# Autodesk Inventor assembly: Robot
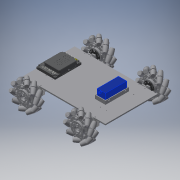
[picture p0: Inventor's stored thumbnail of the model, 180x180]
Saved by Autodesk Inventor 2017 (Build 210142000, 142)
## iProperties
Created: 2017-09-30
Part Number: Robot
Document SubType Name: Assembly
Designer: User
Author: User
## Documents named in this file (6)
- C:\Robotics\CAD\2017-18_CAD\Robot.iam
- C:\Robotics\CAD\2017-18_CAD\PlateFrame1.ipt
- C:\Robotics\CAD\2017-18_CAD\DirectDriveMotorSubAsembly.iam
- C:\Robotics\CAD\COTSParts\Vex\REV-31-1153RevHub.ipt
- C:\Robotics\CAD\2017-18_CAD\batery.ipt
- C:\Robotics\CAD\2017-18_CAD\batteryholder.ipt
## Components (9 placed, 5 different names)
1. PlateFrame1:1 — Mate:1, Mate:2, Mate:3, Mate:4, Mate:6, Mate:7, Mate:8, Mate:11, Mate:12, Mate:14, Mate:15, Mate:16, Mate:17, Mate:21, Mate:22, Mate:26, Mate:27
2. DirectDriveMotorSubAsembly:1 [sub-assembly] — Mate:1, Mate:2, Mate:3
3. DirectDriveMotorSubAsembly:2 [sub-assembly] — Mate:14, Mate:15, Mate:16
4. DirectDriveMotorSubAsembly:3 [sub-assembly] — Mate:11, Mate:12, Mate:17
5. DirectDriveMotorSubAsembly:4 [sub-assembly] — Mate:4, Mate:6, Mate:7, Mate:8
6. REV-31-1153RevHub:1 — Mate:21, Mate:22
7. REV-31-1153RevHub:2 — Mate:27
8. batery:1 — Mate:23, Mate:24, Mate:25
9. batteryholder:1 — Mate:23, Mate:24, Mate:25, Mate:26
## Relationships (20: Mate 20)
- Mate:1: PlateFrame1:1 ↔ DirectDriveMotorSubAsembly:1
- Mate:2: PlateFrame1:1 ↔ DirectDriveMotorSubAsembly:1
- Mate:3: PlateFrame1:1 ↔ DirectDriveMotorSubAsembly:1
- Mate:4: PlateFrame1:1 ↔ DirectDriveMotorSubAsembly:4
- Mate:6: PlateFrame1:1 ↔ DirectDriveMotorSubAsembly:4
- Mate:7: PlateFrame1:1 ↔ DirectDriveMotorSubAsembly:4
- Mate:8: PlateFrame1:1 ↔ DirectDriveMotorSubAsembly:4
- Mate:11: PlateFrame1:1 ↔ DirectDriveMotorSubAsembly:3
- Mate:12: PlateFrame1:1 ↔ DirectDriveMotorSubAsembly:3
- Mate:14: PlateFrame1:1 ↔ DirectDriveMotorSubAsembly:2
- Mate:15: PlateFrame1:1 ↔ DirectDriveMotorSubAsembly:2
- Mate:16: PlateFrame1:1 ↔ DirectDriveMotorSubAsembly:2
- Mate:17: PlateFrame1:1 ↔ DirectDriveMotorSubAsembly:3
- Mate:21: PlateFrame1:1 ↔ REV-31-1153RevHub:1
- Mate:22: PlateFrame1:1 ↔ REV-31-1153RevHub:1
- Mate:23: batery:1 ↔ batteryholder:1
- Mate:24 (3.175 mm): batery:1 ↔ batteryholder:1
- Mate:25 (3.175 mm): batery:1 ↔ batteryholder:1
- Mate:26: PlateFrame1:1 ↔ batteryholder:1
- Mate:27: PlateFrame1:1 ↔ REV-31-1153RevHub:2
